# Autodesk Inventor assembly: DarkPoolFacility
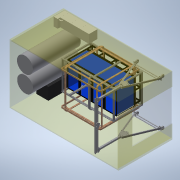
[picture p0: Inventor's stored thumbnail of the model, 180x180]
Saved by Autodesk Inventor 2022 (Build 260153000, 153)
## iProperties
Created: 2021-05-11
Part Number: DarkPoolFacility
Document SubType Name: Assembly
Designer: jamieson-bl
Author: jamieson-bl
## Documents named in this file (12)
- \\Mac\Home\Desktop\WinnipegPMTTestFacility\DarkPoolFacility.iam
- \\Mac\Home\Desktop\WinnipegPMTTestFacility\iManikins\iMan\iMan.iam
- \\Mac\Home\Desktop\WinnipegPMTTestFacility\iManikins\iMandy\iMandy.iam
- \\Mac\Home\Desktop\WinnipegPMTTestFacility\Field Compensation Coils.iam
- \\Mac\Home\Desktop\WinnipegPMTTestFacility\ElectronicsRack.ipt
- \\Mac\Home\Desktop\WinnipegPMTTestFacility\CustomAquariumsStand.ipt
- \\Mac\Home\Desktop\WinnipegPMTTestFacility\CustomAquariumsTank.ipt
- \\Mac\Home\Desktop\WinnipegPMTTestFacility\gantry design\6060gantry.iam
- \\Mac\Home\Desktop\WinnipegPMTTestFacility\Room_0RC039.ipt
- \\Mac\Home\Desktop\WinnipegPMTTestFacility\SumpAssembly.iam
- \\Mac\Home\Desktop\WinnipegPMTTestFacility\3775T610_MOBILE EASY-STORE ADJUSTABLE ALUMINUM CRANE McMaster.ipt
- \\Mac\Home\Desktop\WinnipegPMTTestFacility\CRMI-310VTFWG.ipt
## Components (12 placed, 11 different names)
1. iMan:1 [sub-assembly]
2. iMandy:1 [sub-assembly]
3. Field Compensation Coils:1 [sub-assembly] — Mate:5
4. ElectronicsRack:1 — Mate:13
5. CustomAquariumsStand:1 — Mate:4, Flush:1, Flush:2, Mate:5, Flush:3, Mate:9, Mate:10, Mate:19
6. CustomAquariumsTank:1 — Mate:4, Flush:1, Flush:2, Mate:8
7. 6060gantry:1 [sub-assembly] — Flush:3, Mate:8, Mate:9
8. Room_0RC039:1 — Mate:10, Mate:13, Mate:17, Mate:18, Mate:19, Mate:20, Mate:21
9. SumpAssembly:1 [sub-assembly] — Mate:17
10. 3775T610_MOBILE EASY-STORE ADJUSTABLE ALUMINUM CRANE McMaster:1 — Mate:18
11. CRMI-310VTFWG:1 — Mate:20
12. CRMI-310VTFWG:2 — Mate:21
## Relationships (14: Mate 11, Flush 3)
- Mate:4: CustomAquariumsStand:1 ↔ CustomAquariumsTank:1
- Flush:1: CustomAquariumsStand:1 ↔ CustomAquariumsTank:1
- Flush:2 (15.24 mm): CustomAquariumsStand:1 ↔ CustomAquariumsTank:1
- Mate:5: Field Compensation Coils:1 ↔ CustomAquariumsStand:1
- Flush:3: CustomAquariumsStand:1 ↔ 6060gantry:1
- Mate:8 (40.64 mm): CustomAquariumsTank:1 ↔ 6060gantry:1
- Mate:9 (17.78 mm): CustomAquariumsStand:1 ↔ 6060gantry:1
- Mate:10: CustomAquariumsStand:1 ↔ Room_0RC039:1
- Mate:13: ElectronicsRack:1 ↔ Room_0RC039:1
- Mate:17: Room_0RC039:1 ↔ SumpAssembly:1
- Mate:18 (185.42 mm): Room_0RC039:1 ↔ 3775T610_MOBILE EASY-STORE ADJUSTABLE ALUMINUM CRANE McMaster:1
- Mate:19: CustomAquariumsStand:1 ↔ Room_0RC039:1
- Mate:20: Room_0RC039:1 ↔ CRMI-310VTFWG:1
- Mate:21: Room_0RC039:1 ↔ CRMI-310VTFWG:2
